# Autodesk Inventor assembly: UmlenkrolleHalterEinfach
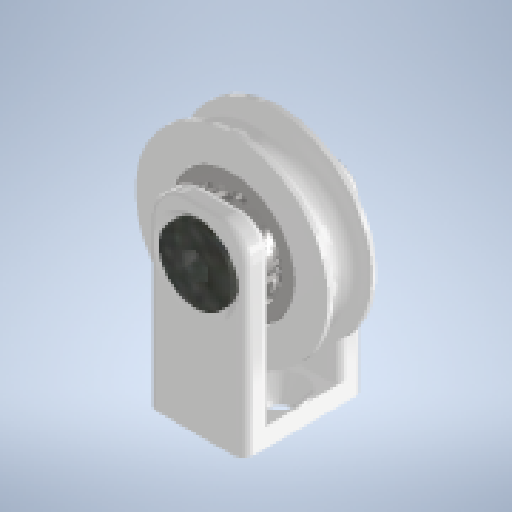
[picture p0: Inventor's stored thumbnail of the model, 512x512]
Saved by Autodesk Inventor 2025 (Build 290162010, 162A)
## iProperties
Created: 2024-11-19
Part Number: UmlenkrolleHalterEinfach
Document SubType Name: Assembly
Designer: Admin
Mass: 6.79388 g
Surface Area: 35.0539 cm^2
Volume: 2.35136 cm^3
Density: 2.88934 g/cm^3
Author: Admin
## Documents named in this file (5)
- C:\Users\Admin\GIT\HDVKBM\CAD\Krandemonstrator\UmlenkrolleHalterEinfach.iam
- C:\Users\Admin\GIT\HDVKBM\CAD\Krandemonstrator\Umlenkrolle.iam
- C:\Users\Admin\GIT\HDVKBM\CAD\Krandemonstrator\HalterUmlenkrolleN.ipt
- C:\Users\Admin\Documents\Inventor\Content Center Files\R2025\de-DE\DIN EN ISO 7089\DIN EN ISO 7089 -  4.ipt
- C:\Users\Admin\Documents\Inventor\Content Center Files\R2025\de-DE\ISO 10642(2)\ISO 10642  - M4  x  12.ipt
## Components (5 placed, 4 different names)
1. HalterUmlenkrolleN:1 — Starr:1
2. Umlenkrolle:1 [sub-assembly] — Drehbar:5
3. DIN EN ISO 10642 M4  x  12:1 — Starr:1
4. DIN EN ISO 7089 4:1
5. DIN EN ISO 7089 4:2 — Drehbar:5
## Relationships (4: RevoluteJoint 3, WeldJoint 1)
- Starr:1 [WeldJoint]: HalterUmlenkrolleN:1 ↔ DIN EN ISO 10642 M4  x  12:1
- [RevoluteJoint]: HalterUmlenkrolleN:1 ↔ DIN EN ISO 7089 4:2
- [RevoluteJoint]: HalterUmlenkrolleN:1 ↔ DIN EN ISO 7089 4:1
- Drehbar:5 [RevoluteJoint]: Umlenkrolle:1 ↔ DIN EN ISO 7089 4:2
